# Autodesk Inventor assembly: kopp_med_adapter
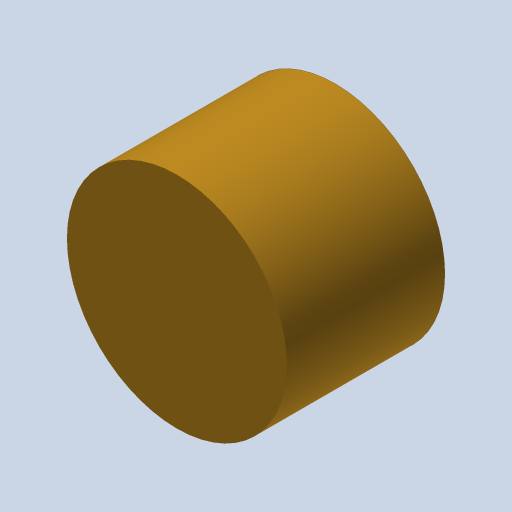
[picture p0: Inventor's stored thumbnail of the model, 512x512]
Saved by Autodesk Inventor 2023.1 (Build 271208000, 208)
## iProperties
Created: 2024-08-14
Part Number: kopp_med_adapter
Document SubType Name: Assembly
Designer: huchonms
Engineer: vikt
Mass: 52.4404 g
Surface Area: 36.924 cm^2
Volume: 6.6803 cm^3
Density: 7.85 g/cm^3
Author: huchonms
Revision Number: 0
tc_part_rev_length: 25
tc_part_rev_width: 18
tc_part_rev_height: 25
tc_part_rev_uom_length: mm
tc_part_rev_volume: 6680
tc_part_rev_uom_volume: mm^3
tc_part_rev_mass: 0.05
tc_part_rev_uom_mass: kg
NOV_FileName: kopp_med_adapter
## Documents named in this file (3)
- C:\VaultWork\Designs\_Scratch_\Marius Huchon\Sommerprosjekt_filer\Heis deler\Actuator_Servo\Inventor\kopp_med_adapter.iam
- C:\VaultWork\Designs\_Scratch_\Marius Huchon\Sommerprosjekt_filer\Heis deler\Heis_kopp.ipt
- C:\VaultWork\Designs\_Scratch_\Marius Huchon\Sommerprosjekt_filer\Heis deler\Actuator_Servo\Inventor\5_grader_adapter.ipt
## Components (2 placed, 2 different names)
1. Heis_kopp:1 — Mate:1
2. 5_grader_adapter:1 — Mate:1
## Relationships (1: Mate 1)
- Mate:1: Heis_kopp:1 ↔ 5_grader_adapter:1
